# Autodesk Inventor assembly: Assembly1
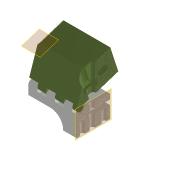
[picture p0: Inventor's stored thumbnail of the model, 180x180]
Saved by Autodesk Inventor 2020 (Build 240168000, 168)
## iProperties
Created: 2020-04-28
Part Number: Assembly1
Document SubType Name: Assembly
Designer: Daniel
Author: Daniel
## Documents named in this file (3)
- F:\Box Sync\DragonVision_DanielKo\Instrumentation\Ephys_rig\Projector_swing v2\Assembly1.iam
- F:\Box Sync\DragonVision_DanielKo\Instrumentation\Ephys_rig\Projector_swing v2\swing.ipt
- F:\Box Sync\DragonVision_DanielKo\Instrumentation\Ephys_rig\Projector_swing v2\anchor.ipt
## Components (2 placed, 2 different names)
1. swing:1 — Flush:1, Mate:1, Angle:1
2. anchor:1 — Flush:1, Mate:1, Angle:1
## Relationships (3: Flush 1, Mate 1, Angle 1)
- Flush:1: swing:1 ↔ anchor:1
- Mate:1: swing:1 ↔ anchor:1
- Angle:1 (162 deg): swing:1 ↔ anchor:1
